# Autodesk Inventor assembly: Box_Assembly
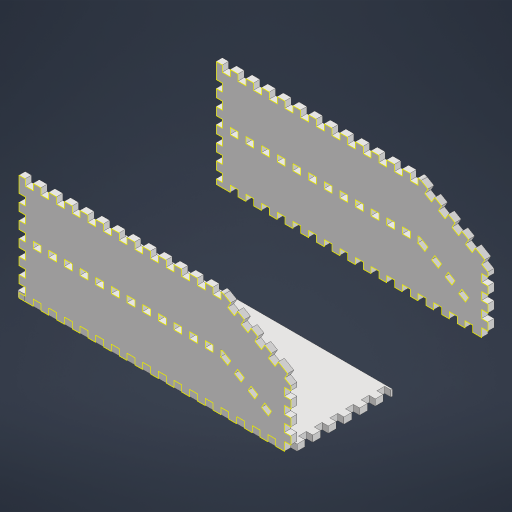
[picture p0: Inventor's stored thumbnail of the model, 512x512]
Saved by Autodesk Inventor 2023 (Build 270158030, 158C)
## iProperties
Created: 2022-06-21
Part Number: Box_Assembly
Document SubType Name: Assembly
Designer: Simon
Author: Simon
## Documents named in this file (3)
- C:\Users\simfe\Desktop\2.Semester\Technische Grundlagen-II\Pixie\3d-modelle\.iam's\Box_Assembly.iam
- C:\Users\simfe\Desktop\2.Semester\Technische Grundlagen-II\Pixie\3d-modelle\.ipt's\SeitenWand.ipt
- C:\Users\simfe\Desktop\2.Semester\Technische Grundlagen-II\Pixie\3d-modelle\.ipt's\BodenWand.ipt
## Components (3 placed, 2 different names)
1. SeitenWand:1 — Mate:1, Flush:1, Flush:2
2. SeitenWand:2 — Mate:1, Flush:1, Flush:2, Mate:2, Mate:3, Mate:4
3. BodenWand:1 — Mate:2, Mate:3, Mate:4
## Relationships (6: Mate 4, Flush 2)
- Mate:1 (122 mm): SeitenWand:1 ↔ SeitenWand:2
- Flush:1: SeitenWand:1 ↔ SeitenWand:2
- Flush:2: SeitenWand:1 ↔ SeitenWand:2
- Mate:2: SeitenWand:2 ↔ BodenWand:1
- Mate:3: SeitenWand:2 ↔ BodenWand:1
- Mate:4: SeitenWand:2 ↔ BodenWand:1
